# Autodesk Inventor assembly: Cuerpo-Rediseno-Ensamble
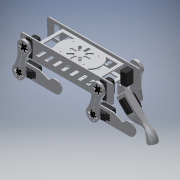
[picture p0: Inventor's stored thumbnail of the model, 180x180]
Saved by Autodesk Inventor 2019 (Build 230136000, 136)
## iProperties
Created: 2020-02-20
Part Number: Cuerpo-Rediseno-Ensamble
Document SubType Name: Assembly
Designer: jacqu
Author: jacqu
## Documents named in this file (8)
- C:\Users\jacqu\Desktop\Robotica1_Proyecto-Cuadrupedo-master\Robotica1-Proyecto_Cuadrupedo\Cuerpo-Rediseno-Ensamble.iam
- C:\Users\jacqu\Desktop\Robotica1_Proyecto-Cuadrupedo-master\Robotica1-Proyecto_Cuadrupedo\Cuerpo - Base.ipt
- C:\Users\jacqu\Desktop\Robotica1_Proyecto-Cuadrupedo-master\Robotica1-Proyecto_Cuadrupedo\Cuerpo - LateralPrueba.ipt
- C:\Users\jacqu\Desktop\Robotica1_Proyecto-Cuadrupedo-master\Robotica1-Proyecto_Cuadrupedo\Pata - Ensamble.iam
- C:\Users\jacqu\Desktop\Robotica1_Proyecto-Cuadrupedo-master\Robotica1-Proyecto_Cuadrupedo\Pata - Ensamble_Lado_Izq.iam
- C:\Users\jacqu\Desktop\Robotica1_Proyecto-Cuadrupedo-master\Robotica1-Proyecto_Cuadrupedo\MG_996R.iam
- C:\Users\jacqu\Desktop\Robotica1_Proyecto-Cuadrupedo-master\Robotica1-Proyecto_Cuadrupedo\Pata - Antebrazo.ipt
- C:\Users\jacqu\Desktop\Robotica1_Proyecto-Cuadrupedo-master\Robotica1-Proyecto_Cuadrupedo\Pata - Brazo - Impresión 3D.ipt
## Components (12 placed, 7 different names)
1. Cuerpo - Base:1 — Mate:7, Mate:8, Mate:16
2. Cuerpo - LateralPrueba:1 — Mate:1, Mate:2, Mate:3, Mate:4, Mate:5, Mate:6, Mate:7, Mate:8, Mate:11, Mate:12, Mate:15, Mate:16, Mate:17
3. Pata - Ensamble:1 [sub-assembly] — Mate:1, Mate:2, Mate:3
4. Cuerpo - Base:2 — Mate:11, Mate:12, Mate:13, Mate:14, Mate:15
5. Pata - Ensamble:2 [sub-assembly] — Mate:4, Mate:5, Mate:6
6. Cuerpo - LateralPrueba:2 — Mate:13, Mate:14, Mate:17, Mate:18, Mate:19, Mate:20, Mate:21, Mate:22, Mate:23, Coincidencia:24, Coincidencia:25, Coincidencia:26
7. Pata - Ensamble_Lado_Izq:1 [sub-assembly] — Mate:18, Mate:20, Mate:23
8. Pata - Ensamble_Lado_Izq:2 [sub-assembly] — Mate:19, Mate:21, Mate:22
9. MG_996R:1 [sub-assembly] — Coincidencia:24, Coincidencia:25, Coincidencia:26, Coincidencia:27, Coincidencia:28
10. Pata - Antebrazo:1 — Coincidencia:27, Coincidencia:28, Coincidencia:29, Coincidencia:30
11. MG_996R:2 [sub-assembly] — Coincidencia:29, Coincidencia:30, Coincidencia:31, Coincidencia:32, Coincidencia:33
12. Pata - Brazo - Impresión 3D:1 — Coincidencia:31, Coincidencia:32, Coincidencia:33
## Relationships (31: Mate 31)
- Mate:1: Cuerpo - LateralPrueba:1 ↔ Pata - Ensamble:1
- Mate:2: Cuerpo - LateralPrueba:1 ↔ Pata - Ensamble:1
- Mate:3: Cuerpo - LateralPrueba:1 ↔ Pata - Ensamble:1
- Mate:4: Cuerpo - LateralPrueba:1 ↔ Pata - Ensamble:2
- Mate:5: Cuerpo - LateralPrueba:1 ↔ Pata - Ensamble:2
- Mate:6: Cuerpo - LateralPrueba:1 ↔ Pata - Ensamble:2
- Mate:7: Cuerpo - Base:1 ↔ Cuerpo - LateralPrueba:1
- Mate:8: Cuerpo - Base:1 ↔ Cuerpo - LateralPrueba:1
- Mate:11: Cuerpo - LateralPrueba:1 ↔ Cuerpo - Base:2
- Mate:12: Cuerpo - LateralPrueba:1 ↔ Cuerpo - Base:2
- Mate:13: Cuerpo - Base:2 ↔ Cuerpo - LateralPrueba:2
- Mate:14: Cuerpo - Base:2 ↔ Cuerpo - LateralPrueba:2
- Mate:15 (-3.3 mm): Cuerpo - LateralPrueba:1 ↔ Cuerpo - Base:2
- Mate:16 (-3.3 mm): Cuerpo - Base:1 ↔ Cuerpo - LateralPrueba:1
- Mate:17 (83.3 mm): Cuerpo - LateralPrueba:1 ↔ Cuerpo - LateralPrueba:2
- Mate:18: Cuerpo - LateralPrueba:2 ↔ Pata - Ensamble_Lado_Izq:1
- Mate:19: Cuerpo - LateralPrueba:2 ↔ Pata - Ensamble_Lado_Izq:2
- Mate:20: Cuerpo - LateralPrueba:2 ↔ Pata - Ensamble_Lado_Izq:1
- Mate:21: Cuerpo - LateralPrueba:2 ↔ Pata - Ensamble_Lado_Izq:2
- Mate:22: Cuerpo - LateralPrueba:2 ↔ Pata - Ensamble_Lado_Izq:2
- Mate:23: Cuerpo - LateralPrueba:2 ↔ Pata - Ensamble_Lado_Izq:1
- Coincidencia:24 [Mate]: Cuerpo - LateralPrueba:2 ↔ MG_996R:1
- Coincidencia:25 [Mate]: Cuerpo - LateralPrueba:2 ↔ MG_996R:1
- Coincidencia:26 [Mate]: Cuerpo - LateralPrueba:2 ↔ MG_996R:1
- Coincidencia:27 [Mate]: MG_996R:1 ↔ Pata - Antebrazo:1
- Coincidencia:28 [Mate]: MG_996R:1 ↔ Pata - Antebrazo:1
- Coincidencia:29 [Mate]: Pata - Antebrazo:1 ↔ MG_996R:2
- Coincidencia:30 [Mate]: Pata - Antebrazo:1 ↔ MG_996R:2
- Coincidencia:31 [Mate]: MG_996R:2 ↔ Pata - Brazo - Impresión 3D:1
- Coincidencia:32 [Mate]: MG_996R:2 ↔ Pata - Brazo - Impresión 3D:1
- Coincidencia:33 [Mate]: MG_996R:2 ↔ Pata - Brazo - Impresión 3D:1
## Named parameters: sa_0 = 2.05244, sa_1 = -444.817, sa_2 = -4.44822e-13
note: some values were not read from the file. Shown as the stored number, unit unknown: "sa_0", "sa_1", "sa_2".
